# Autodesk Inventor assembly: REV Single Stage Spur Gearbox (REV-21-2099)
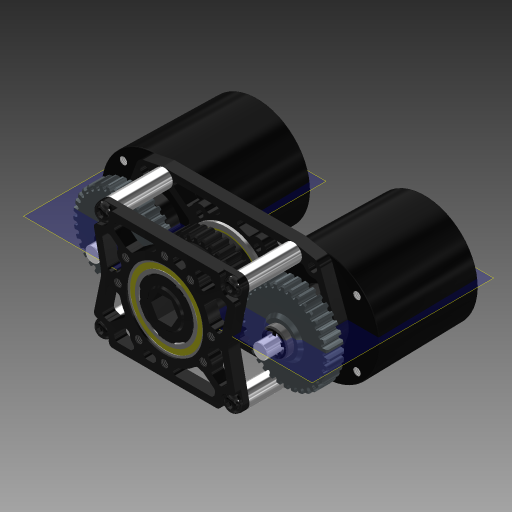
[picture p0: Inventor's stored thumbnail of the model, 512x512]
Saved by Autodesk Inventor 2023 (Build 270158030, 158C)
## iProperties
Created: 2023-01-27
Part Number: REV Single Stage Spur Gearbox (REV-21-2099)
Document SubType Name: Assembly
Designer: Max Boord
Author: Max Boord
## iProperties of the stored document MemberDocs/x5qqfnf21Mkmzj5t2D2kvyo4fUf
Created: 2023-01-27
Part Number: REV Single Stage Spur Gearbox (REV-21-2099)
Document SubType Name: Assembly
Designer: Max Boord
Author: Max Boord
## iProperties of the stored document MemberDocs/x4j3nuzvhLswg2ana1jbnmmlkNg
Created: 2023-01-27
Part Number: REV Single Stage Spur Gearbox (REV-21-2099)
Document SubType Name: Assembly
Designer: Max Boord
Author: Max Boord
## iProperties of the stored document MemberDocs/xFzuzt52mAc0nw02eKli1b5xy5h
Created: 2023-01-27
Part Number: REV Single Stage Spur Gearbox (REV-21-2099)
Document SubType Name: Assembly
Designer: Max Boord
Author: Max Boord
## iProperties of the stored document MemberDocs/xBnqqbpf1Bszva0ll5ieladu5Xf
Created: 2023-01-27
Part Number: REV Single Stage Spur Gearbox (REV-21-2099)
Document SubType Name: Assembly
Designer: Max Boord
Author: Max Boord
## iProperties of the stored document MemberDocs/xQfox2mnrPslwk2vmKgohnjx01b
Created: 2023-01-27
Part Number: REV Single Stage Spur Gearbox (REV-21-2099)
Document SubType Name: Assembly
Designer: Max Boord
Author: Max Boord
## iProperties of the stored document MemberDocs/xYvkiv4wzAkae221eUxm53huiEh
Created: 2023-01-27
Part Number: REV Single Stage Spur Gearbox (REV-21-2099)
Document SubType Name: Assembly
Designer: Max Boord
Author: Max Boord
## Documents named in this file (30)
- D:\Collaborative Robots\COTS Parts\General Gearboxes\COTS Gearboxes\REV Single Stage Spur Gearbox (REV-21-2099)\REV Single Stage Spur Gearbox (REV-21-2099).iam
- D:\Collaborative Robots\COTS Parts\General Gearboxes\COTS Gearboxes\REV Single Stage Spur Gearbox (REV-21-2099)\REV Single Stage Spur Gearbox Back Plate (REV-21-2099-P01).ipt
- D:\Collaborative Robots\COTS Parts\General Gearboxes\COTS Gearboxes\REV Single Stage Spur Gearbox (REV-21-2099)\REV Single Stage Spur Gearbox MAXSpline Adaptor (REV-21-2079).ipt
- D:\Collaborative Robots\COTS Parts\General Gearboxes\COTS Gearboxes\REV Single Stage Spur Gearbox (REV-21-2099)\REV Single Stage Spur Gearbox Front Plate (REV-21-2099-P02).ipt
- D:\Collaborative Robots\COTS Parts\Power Transfer\Bearings and Bushings\Bearings\F6806ZZ.ipt
- D:\Collaborative Robots\COTS Parts\Power Transfer\Bearings and Bushings\Bearings.ipt
- D:\Collaborative Robots\COTS Parts\Hardware\Spacers\Spacers & Standoffs\Aluminum Unthreaded Spacer (No. 10 x 1.125Lg x 0.375OD).ipt
- D:\Collaborative Robots\COTS Parts\Hardware\Spacers\Spacers & Standoffs.ipt
- D:\Collaborative Robots\COTS Parts\Hardware\Spacers\MAXSpline Spacers.ipt
- D:\Collaborative Robots\COTS Parts\General Gearboxes\COTS Gearboxes\REV Single Stage Spur Gearbox (REV-21-2099)\36T REV 500 Hex Gear (REV-21-1929).ipt
- D:\Collaborative Robots\COTS Parts\General Gearboxes\COTS Gearboxes\REV Single Stage Spur Gearbox (REV-21-2099)\36T MAXSpline Gear (REV-21-3012).ipt
- D:\Collaborative Robots\COTS Parts\Hardware\Fasteners\Machine Screws\10-32 UNFx1.5 Button Head Cap Screw.ipt
- D:\Collaborative Robots\COTS Parts\Hardware\Fasteners\Machine Screws.ipt
- D:\Collaborative Robots\COTS Parts\Power Transfer\Adaptors and Couplers\8mm to 1_2_ Hex Adapter (217-3255).ipt
- D:\Collaborative Robots\COTS Parts\Motors\FRC\NEO.ipt
- D:\Collaborative Robots\COTS Parts\Power Transfer\Adaptors and Couplers\8mm to 500 Hex Adapter.ipt
- D:\Collaborative Robots\COTS Parts\Hardware\Spacers\REV Thin Hex Spacers.ipt
- D:\Collaborative Robots\COTS Parts\Hardware\Spacers\REV CIM Motor Shaft Spacer (REV-21-2078).ipt
- D:\Collaborative Robots\COTS Parts\Hardware\Fasteners\8mm CIM Shaft Retaining Ring.ipt
- D:\Collaborative Robots\COTS Parts\General Gearboxes\COTS Gearboxes\REV Single Stage Spur Gearbox (REV-21-2099)\24T REV 500 Hex Gear (REV-21-1923).ipt
- D:\Collaborative Robots\COTS Parts\General Gearboxes\COTS Gearboxes\REV Single Stage Spur Gearbox (REV-21-2099)\48T MAXSpline Gear (REV-21-3018).ipt
- D:\Collaborative Robots\COTS Parts\General Gearboxes\COTS Gearboxes\REV Single Stage Spur Gearbox (REV-21-2099)\54T MAXSpline Gear (REV-21-3021).ipt
- D:\Collaborative Robots\COTS Parts\General Gearboxes\COTS Gearboxes\REV Single Stage Spur Gearbox (REV-21-2099)\18T REV 500 Hex Gear (REV-21-1920).ipt
- D:\Collaborative Robots\COTS Parts\Hardware\Fasteners\Machine Screws\10-32 UNFx0.5 Button Head Cap Screw.ipt
- D:\Collaborative Robots\COTS Parts\General Gearboxes\Planetaries\Versaplanetary V2\Versaplanetary Generator V2\2 stage 775 input, .5(_DQ) Hex output.iam
- D:\Collaborative Robots\COTS Parts\General Gearboxes\Planetaries\Versaplanetary V2\Versaplanetary Generator V2.iam
- D:\Collaborative Robots\COTS Parts\Hardware\Fasteners\Washers\Washer 0.265ID 0.688OD 0.055Thick.ipt
- D:\Collaborative Robots\COTS Parts\Hardware\Fasteners\Washers.ipt
- D:\Collaborative Robots\COTS Parts\Hardware\Fasteners\Machine Screws\1(_FS)4-20 UNCx0.5 Button Head Cap Screw.ipt
- D:\Collaborative Robots\COTS Parts\General Gearboxes\Planetaries\Maxplanatery\MAXPlanetary.iam
## Components (36 placed, 19 different names)
1. REV Single Stage Spur Gearbox Back Plate (REV-21-2099-P01):1 — Insert:1, Mate:2, Insert:7, Mate:3, Mate:4, Mate:5, Insert:17, Insert:18
2. REV Single Stage Spur Gearbox MAXSpline Adaptor (REV-21-2079):1 — Insert:8
3. REV Single Stage Spur Gearbox Front Plate (REV-21-2099-P02):1 — Insert:2, Insert:3, Insert:4, Insert:5, Insert:6, Flush:1, Flush:2, Insert:13, Insert:14, Insert:15, Insert:16
4. F6806ZZ:1 — Insert:1, Mate:1, Insert:9
5. F6806ZZ:2 — Insert:2, Mate:1, Insert:8, Insert:11
6. Aluminum Unthreaded Spacer (No. 10 x 1.125Lg x 0.375OD):1 — Insert:4
7. Aluminum Unthreaded Spacer (No. 10 x 1.125Lg x 0.375OD):2 — Insert:6
8. Aluminum Unthreaded Spacer (No. 10 x 1.125Lg x 0.375OD):3 — Insert:5
9. Aluminum Unthreaded Spacer (No. 10 x 1.125Lg x 0.375OD):4 — Insert:3, Mate:2, Insert:7
10. MAXSpline Spacers:1 — Insert:9, Insert:10, Insert:28, Insert:32
11. 36T REV 500 Hex Gear (REV-21-1929):1 — Flush:4, Mate:5
12. 36T MAXSpline Gear (REV-21-3012):1 — Insert:10
13. MAXSpline Spacers:2 — Insert:12
14. MAXSpline Spacers:3 — Insert:11, Insert:12
15. 36T REV 500 Hex Gear (REV-21-1929):2 — Flush:4, Mate:4, Insert:23
16. 10-32 UNFx1.5 Button Head Cap Screw:1 — Insert:16
17. 10-32 UNFx1.5 Button Head Cap Screw:2 — Insert:13
18. 10-32 UNFx1.5 Button Head Cap Screw:3 — Insert:14
19. 10-32 UNFx1.5 Button Head Cap Screw:4 — Insert:15
20. 8mm to 1_2_ Hex Adapter (217-3255):2
21. NEO:1 — Insert:17, Insert:21
22. NEO:2 — Insert:18, Insert:20, Insert:30
23. 8mm to 500 Hex Adapter:1 — Insert:21, Insert:22, Insert:26
24. 8mm to 500 Hex Adapter:2 — Insert:20, Insert:27
25. REV Thin Hex Spacers:1 — Insert:22, Insert:23, Insert:29, Insert:33
26. REV CIM Motor Shaft Spacer (REV-21-2078):1 — Insert:25, Insert:26
27. REV CIM Motor Shaft Spacer (REV-21-2078):2 — Insert:24, Insert:27
28. 8mm CIM Shaft Retaining Ring:1 — Insert:25
29. 8mm CIM Shaft Retaining Ring:2 — Insert:24
30. 24T REV 500 Hex Gear (REV-21-1923):1 — Insert:29
31. 48T MAXSpline Gear (REV-21-3018):1 — Insert:28
32. 24T REV 500 Hex Gear (REV-21-1923):2 — Insert:31
33. REV Thin Hex Spacers:2 — Insert:30, Insert:31, Insert:34
34. 54T MAXSpline Gear (REV-21-3021):1 — Insert:32
35. 18T REV 500 Hex Gear (REV-21-1920):1 — Flush:5, Insert:33
36. 18T REV 500 Hex Gear (REV-21-1920):2 — Flush:5, Insert:34
## Relationships (42: Insert 33, Mate 5, Flush 4)
- Insert:1: REV Single Stage Spur Gearbox Back Plate (REV-21-2099-P01):1 ↔ F6806ZZ:1
- Insert:2: REV Single Stage Spur Gearbox Front Plate (REV-21-2099-P02):1 ↔ F6806ZZ:2
- Insert:3: REV Single Stage Spur Gearbox Front Plate (REV-21-2099-P02):1 ↔ Aluminum Unthreaded Spacer (No. 10 x 1.125Lg x 0.375OD):4
- Insert:4: REV Single Stage Spur Gearbox Front Plate (REV-21-2099-P02):1 ↔ Aluminum Unthreaded Spacer (No. 10 x 1.125Lg x 0.375OD):1
- Insert:5: REV Single Stage Spur Gearbox Front Plate (REV-21-2099-P02):1 ↔ Aluminum Unthreaded Spacer (No. 10 x 1.125Lg x 0.375OD):3
- Insert:6: REV Single Stage Spur Gearbox Front Plate (REV-21-2099-P02):1 ↔ Aluminum Unthreaded Spacer (No. 10 x 1.125Lg x 0.375OD):2
- Mate:1: F6806ZZ:1 ↔ F6806ZZ:2
- Mate:2: REV Single Stage Spur Gearbox Back Plate (REV-21-2099-P01):1 ↔ Aluminum Unthreaded Spacer (No. 10 x 1.125Lg x 0.375OD):4
- Insert:7: REV Single Stage Spur Gearbox Back Plate (REV-21-2099-P01):1 ↔ Aluminum Unthreaded Spacer (No. 10 x 1.125Lg x 0.375OD):4
- Insert:8: REV Single Stage Spur Gearbox MAXSpline Adaptor (REV-21-2079):1 ↔ F6806ZZ:2
- Insert:9: F6806ZZ:1 ↔ MAXSpline Spacers:1
- Insert:10: MAXSpline Spacers:1 ↔ 36T MAXSpline Gear (REV-21-3012):1
- Insert:11: F6806ZZ:2 ↔ MAXSpline Spacers:3
- Insert:12: MAXSpline Spacers:2 ↔ MAXSpline Spacers:3
- Mate:3: REV Single Stage Spur Gearbox Back Plate (REV-21-2099-P01):1
- Flush:1: REV Single Stage Spur Gearbox Front Plate (REV-21-2099-P02):1
- Flush:2: REV Single Stage Spur Gearbox Front Plate (REV-21-2099-P02):1
- Insert:13: REV Single Stage Spur Gearbox Front Plate (REV-21-2099-P02):1 ↔ 10-32 UNFx1.5 Button Head Cap Screw:2
- Insert:14: REV Single Stage Spur Gearbox Front Plate (REV-21-2099-P02):1 ↔ 10-32 UNFx1.5 Button Head Cap Screw:3
- Insert:15: REV Single Stage Spur Gearbox Front Plate (REV-21-2099-P02):1 ↔ 10-32 UNFx1.5 Button Head Cap Screw:4
- Insert:16: REV Single Stage Spur Gearbox Front Plate (REV-21-2099-P02):1 ↔ 10-32 UNFx1.5 Button Head Cap Screw:1
- Flush:4: 36T REV 500 Hex Gear (REV-21-1929):1 ↔ 36T REV 500 Hex Gear (REV-21-1929):2
- Mate:4: REV Single Stage Spur Gearbox Back Plate (REV-21-2099-P01):1 ↔ 36T REV 500 Hex Gear (REV-21-1929):2
- Mate:5: REV Single Stage Spur Gearbox Back Plate (REV-21-2099-P01):1 ↔ 36T REV 500 Hex Gear (REV-21-1929):1
- Insert:17: REV Single Stage Spur Gearbox Back Plate (REV-21-2099-P01):1 ↔ NEO:1
- Insert:18: REV Single Stage Spur Gearbox Back Plate (REV-21-2099-P01):1 ↔ NEO:2
- Insert:20: NEO:2 ↔ 8mm to 500 Hex Adapter:2
- Insert:21: NEO:1 ↔ 8mm to 500 Hex Adapter:1
- Insert:22 (-0.95 mm): 8mm to 500 Hex Adapter:1 ↔ REV Thin Hex Spacers:1
- Insert:23: 36T REV 500 Hex Gear (REV-21-1929):2 ↔ REV Thin Hex Spacers:1
- Insert:24: REV CIM Motor Shaft Spacer (REV-21-2078):2 ↔ 8mm CIM Shaft Retaining Ring:2
- Insert:25: REV CIM Motor Shaft Spacer (REV-21-2078):1 ↔ 8mm CIM Shaft Retaining Ring:1
- Insert:26: 8mm to 500 Hex Adapter:1 ↔ REV CIM Motor Shaft Spacer (REV-21-2078):1
- Insert:27: 8mm to 500 Hex Adapter:2 ↔ REV CIM Motor Shaft Spacer (REV-21-2078):2
- Insert:28: MAXSpline Spacers:1 ↔ 48T MAXSpline Gear (REV-21-3018):1
- Insert:29: REV Thin Hex Spacers:1 ↔ 24T REV 500 Hex Gear (REV-21-1923):1
- Insert:30 (0.95 mm): NEO:2 ↔ REV Thin Hex Spacers:2
- Insert:31: 24T REV 500 Hex Gear (REV-21-1923):2 ↔ REV Thin Hex Spacers:2
- Insert:32: MAXSpline Spacers:1 ↔ 54T MAXSpline Gear (REV-21-3021):1
- Flush:5: 18T REV 500 Hex Gear (REV-21-1920):1 ↔ 18T REV 500 Hex Gear (REV-21-1920):2
- Insert:33: REV Thin Hex Spacers:1 ↔ 18T REV 500 Hex Gear (REV-21-1920):1
- Insert:34: REV Thin Hex Spacers:2 ↔ 18T REV 500 Hex Gear (REV-21-1920):2
